# Autodesk Inventor assembly: MXQ12-40AS-M9B
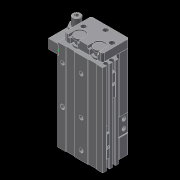
[picture p0: Inventor's stored thumbnail of the model, 180x180]
Saved by Autodesk Inventor 2021.1 (Build 251245000, 245)
## iProperties
Created: 2008-11-14
Part Number: MXQ12-40AS-M9B
Document SubType Name: Assembly
変換規格: STEP AP214IS
ファイル名: MXMXQ121113230155334.step
プリプロセッサ: SolidWorks 2009
ポストプロセッサ: Build: 342, Release: 2008 SP3 - Date: Tue 05/27/2008
送信済み単位: MILLIMETERS
不明: 1e-05
Title: エアスライドテーブル
## Documents named in this file (6)
- Z:\inventorroom\sample\unit4\MXQ12-40AS\MXQ12-40AS-M9B.iam
- Z:\inventorroom\sample\unit4\MXQ12-40AS\MXQ12-40AS-M9B.step_A9+F9_M9B.iam
- Z:\inventorroom\sample\unit4\MXQ12-40AS\MXQ12-40AS-M9B.step_ExtensionEnd_12A.iam
- Z:\inventorroom\sample\unit4\MXQ12-40AS\MXQ12-40AS-M9B.step_TableMounting_12A.ipt
- Z:\inventorroom\sample\unit4\MXQ12-40AS\MXQ12-40AS-M9B.step_MXQ3149Tube_12-40.ipt
- Z:\inventorroom\sample\unit4\MXQ12-40AS\MXQ12-40AS-M9B.step_MXQTables_12-40.ipt
## Components (6 placed, 5 different names)
1. MXQ12-40AS-M9B.step_A9+F9_M9B:1 [sub-assembly]
2. MXQ12-40AS-M9B.step_ExtensionEnd_12A:1 [sub-assembly]
3. MXQ12-40AS-M9B.step_TableMounting_12A:1 — フラッシュ:1, フラッシュ:2, フラッシュ:3
4. MXQ12-40AS-M9B.step_A9+F9_M9B:2 [sub-assembly]
5. MXQ12-40AS-M9B.step_MXQ3149Tube_12-40:1 — フラッシュ:4, フラッシュ:5, 1
6. MXQ12-40AS-M9B.step_MXQTables_12-40:1 — フラッシュ:1, フラッシュ:2, フラッシュ:3, フラッシュ:4, フラッシュ:5, 1
## Relationships (6: Flush 6)
- フラッシュ:1 [Flush] (0.6 mm): MXQ12-40AS-M9B.step_TableMounting_12A:1 ↔ MXQ12-40AS-M9B.step_MXQTables_12-40:1
- フラッシュ:2 [Flush] (11.7 mm): MXQ12-40AS-M9B.step_TableMounting_12A:1 ↔ MXQ12-40AS-M9B.step_MXQTables_12-40:1
- フラッシュ:3 [Flush] (19 mm): MXQ12-40AS-M9B.step_TableMounting_12A:1 ↔ MXQ12-40AS-M9B.step_MXQTables_12-40:1
- フラッシュ:4 [Flush] (4.5 mm): MXQ12-40AS-M9B.step_MXQ3149Tube_12-40:1 ↔ MXQ12-40AS-M9B.step_MXQTables_12-40:1
- フラッシュ:5 [Flush] (12 mm): MXQ12-40AS-M9B.step_MXQ3149Tube_12-40:1 ↔ MXQ12-40AS-M9B.step_MXQTables_12-40:1
- 1 [Flush] (1 mm): MXQ12-40AS-M9B.step_MXQ3149Tube_12-40:1 ↔ MXQ12-40AS-M9B.step_MXQTables_12-40:1
